# Autodesk Inventor assembly: LineSensorUnit
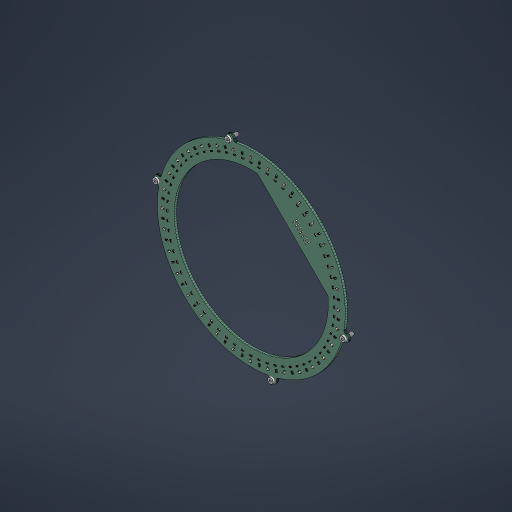
[picture p0: Inventor's stored thumbnail of the model, 512x512]
Saved by Autodesk Inventor 2024.2 (Build 282272000, 272)
## iProperties
Created: 2024-01-10
Part Number: LineSensorUnit
Document SubType Name: Assembly
Designer: Hanaoka
Author: Hanaoka
## Documents named in this file (4)
- G:\共有ドライブ\reRo\05_個人\hanaoka\inventor\PCBs\LineSensorUnit.iam
- G:\共有ドライブ\reRo\05_個人\hanaoka\inventor\PCBs\LineSensor_v2\LineSensor_v2.iam
- G:\共有ドライブ\reRo\05_個人\hanaoka\inventor\PCBs\LineSensor_PCB.ipt
- G:\共有ドライブ\reRo\05_個人\hanaoka\inventor\Screw\M2xL6\M2x6.ipt
## Components (6 placed, 3 different names)
1. LineSensor_v2:1 [sub-assembly] — フラッシュ:2, フラッシュ:1, 正接:1
2. LineSensor_PCB:1 — フラッシュ:2, フラッシュ:1, 正接:1, 挿入:1, 挿入:2, 挿入:3, 挿入:4
3. M2x6:1 — 挿入:1
4. M2x6:2 — 挿入:3
5. M2x6:3 — 挿入:4
6. M2x6:4 — 挿入:2
## Relationships (7: Insert 4, Flush 2, Tangent 1)
- フラッシュ:2 [Flush]: LineSensor_v2:1 ↔ LineSensor_PCB:1
- フラッシュ:1 [Flush]: LineSensor_v2:1 ↔ LineSensor_PCB:1
- 正接:1 [Tangent]: LineSensor_v2:1 ↔ LineSensor_PCB:1
- 挿入:1 [Insert] (0.5 mm): LineSensor_PCB:1 ↔ M2x6:1
- 挿入:2 [Insert] (0.5 mm): LineSensor_PCB:1 ↔ M2x6:4
- 挿入:3 [Insert] (0.5 mm): LineSensor_PCB:1 ↔ M2x6:2
- 挿入:4 [Insert] (0.5 mm): LineSensor_PCB:1 ↔ M2x6:3
